# Autodesk Inventor assembly: base
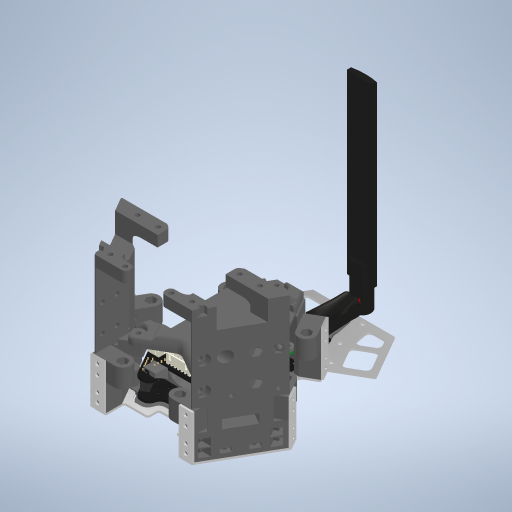
[picture p0: Inventor's stored thumbnail of the model, 512x512]
Saved by Autodesk Inventor 2024.1 (Build 281209000, 209)
## iProperties
Created: 2025-02-03
Part Number: base
Document SubType Name: Assembly
Designer: hibik
Author: hibik
## Documents named in this file (11)
- C:\Users\hibik\Documents\Robomech\RESCUE\ORCA\hard\flame_base\base.iam
- C:\Users\hibik\Documents\Robomech\RESCUE\ORCA\hard\flame_base\base_plate.ipt
- C:\Users\hibik\Documents\Robomech\RESCUE\ORCA\hard\flame_base\base_plate_towheel.ipt
- C:\Users\hibik\Documents\Robomech\RESCUE\ORCA\hard\flame_base\base_plate_towheel_front_right.ipt
- C:\Users\hibik\Documents\Robomech\RESCUE\ORCA\hard\std_parts\Buffalo_Wl-U2-433DHP.ipt
- C:\Users\hibik\Documents\Robomech\RESCUE\ORCA\hard\board\CORE_model\external_io_usbA.iam
- C:\Users\hibik\Documents\Robomech\RESCUE\ORCA\hard\flame_base\base_plate_towheel_front_right_MIR.ipt
- C:\Users\hibik\Documents\Robomech\RESCUE\ORCA\hard\flame_base\Assy_CORE_board.iam
- C:\Users\hibik\Documents\Robomech\RESCUE\ORCA\hard\omni_wheel\wheel_setter_plate.ipt
- C:\Users\hibik\Documents\Robomech\RESCUE\ORCA\hard\omni_wheel\wheel_setter.ipt
- C:\Users\hibik\Documents\Robomech\RESCUE\ORCA\hard\flame_base\CORE_board_cover.ipt
## Components (17 placed, 10 different names)
1. base_plate:1 — 挿入:1, 挿入:2, フラッシュ:9, フラッシュ:10, メイト:1, 角度:2
2. base_plate_towheel:3 — フラッシュ:9, フラッシュ:10, メイト:1, 挿入:5, 角度:1, 挿入:8, 挿入:9, 挿入:17, 挿入:18
3. base_plate_towheel_front_right:1 — 挿入:1, 挿入:2, 挿入:6, 挿入:7, 挿入:10, 挿入:11, 挿入:12
4. Buffalo_Wl-U2-433DHP:1 — メイト:2, メイト:3, フラッシュ:11
5. external_io_usbA:1 [sub-assembly] — 挿入:5, 角度:1, メイト:2, メイト:3
6. base_plate_towheel_front_right_MIR:1 — 挿入:13, 挿入:14, 挿入:15, 挿入:16, 挿入:25
7. Assy_CORE_board:1 [sub-assembly] — 挿入:6, 角度:2
8. wheel_setter_plate:1 — 挿入:7, 挿入:10, 挿入:23, 挿入:24
9. wheel_setter_plate:2 — 挿入:8, 挿入:9
10. wheel_setter_plate:3 — 挿入:17, 挿入:18, 挿入:19, 挿入:20
11. wheel_setter_plate:4 — 挿入:15, 挿入:16
12. wheel_setter_plate:5 — 挿入:13, 挿入:14, 挿入:21, 挿入:22
13. wheel_setter_plate:6 — 挿入:11, 挿入:12
14. wheel_setter:1 — 挿入:19, 挿入:20
15. wheel_setter:2 — 挿入:23, 挿入:24
16. wheel_setter:3 — 挿入:21, 挿入:22
17. CORE_board_cover:1 — 挿入:25, 角度:3
## Relationships (32: Insert 23, Flush 3, Mate 3, Angle 3)
- 挿入:1 [Insert]: base_plate:1 ↔ base_plate_towheel_front_right:1
- 挿入:2 [Insert]: base_plate:1 ↔ base_plate_towheel_front_right:1
- フラッシュ:9 [Flush]: base_plate:1 ↔ base_plate_towheel:3
- フラッシュ:10 [Flush]: base_plate:1 ↔ base_plate_towheel:3
- メイト:1 [Mate]: base_plate:1 ↔ base_plate_towheel:3
- 挿入:5 [Insert] (0.5 mm): base_plate_towheel:3 ↔ external_io_usbA:1
- 角度:1 [Angle] (0 deg): base_plate_towheel:3 ↔ external_io_usbA:1
- メイト:2 [Mate] (2 mm): Buffalo_Wl-U2-433DHP:1 ↔ external_io_usbA:1
- メイト:3 [Mate] (0.5 mm): Buffalo_Wl-U2-433DHP:1 ↔ external_io_usbA:1
- フラッシュ:11 [Flush]: Buffalo_Wl-U2-433DHP:1
- 挿入:6 [Insert]: base_plate_towheel_front_right:1 ↔ Assy_CORE_board:1
- 角度:2 [Angle] (0 deg): base_plate:1 ↔ Assy_CORE_board:1
- 挿入:7 [Insert]: base_plate_towheel_front_right:1 ↔ wheel_setter_plate:1
- 挿入:8 [Insert]: base_plate_towheel:3 ↔ wheel_setter_plate:2
- 挿入:9 [Insert]: base_plate_towheel:3 ↔ wheel_setter_plate:2
- 挿入:10 [Insert]: base_plate_towheel_front_right:1 ↔ wheel_setter_plate:1
- 挿入:11 [Insert]: base_plate_towheel_front_right:1 ↔ wheel_setter_plate:6
- 挿入:12 [Insert]: base_plate_towheel_front_right:1 ↔ wheel_setter_plate:6
- 挿入:13 [Insert]: base_plate_towheel_front_right_MIR:1 ↔ wheel_setter_plate:5
- 挿入:14 [Insert]: base_plate_towheel_front_right_MIR:1 ↔ wheel_setter_plate:5
- 挿入:15 [Insert]: base_plate_towheel_front_right_MIR:1 ↔ wheel_setter_plate:4
- 挿入:16 [Insert]: base_plate_towheel_front_right_MIR:1 ↔ wheel_setter_plate:4
- 挿入:17 [Insert]: base_plate_towheel:3 ↔ wheel_setter_plate:3
- 挿入:18 [Insert]: base_plate_towheel:3 ↔ wheel_setter_plate:3
- 挿入:19 [Insert]: wheel_setter_plate:3 ↔ wheel_setter:1
- 挿入:20 [Insert]: wheel_setter_plate:3 ↔ wheel_setter:1
- 挿入:21 [Insert]: wheel_setter_plate:5 ↔ wheel_setter:3
- 挿入:22 [Insert]: wheel_setter_plate:5 ↔ wheel_setter:3
- 挿入:23 [Insert]: wheel_setter_plate:1 ↔ wheel_setter:2
- 挿入:24 [Insert]: wheel_setter_plate:1 ↔ wheel_setter:2
- 挿入:25 [Insert]: base_plate_towheel_front_right_MIR:1 ↔ CORE_board_cover:1
- 角度:3 [Angle] (0 deg): CORE_board_cover:1
